# Autodesk Inventor assembly: 2.75 Omni AS, No Insert_CPY1
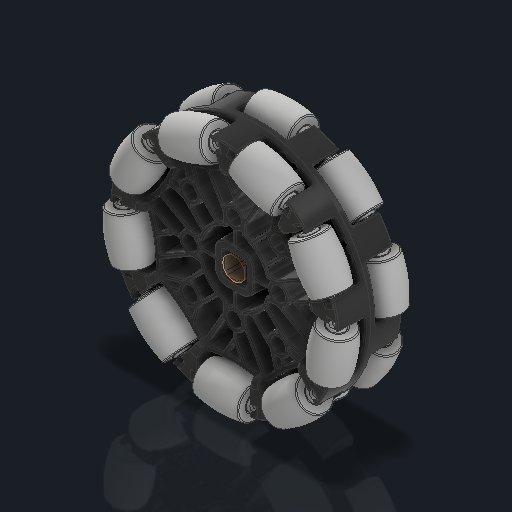
[picture p0: Inventor's stored thumbnail of the model, 512x512]
Saved by Autodesk Inventor 2023.2 (Build 272271030, 271C)
## iProperties
Created: 2022-08-02
Part Number: 2.75 Omni AS, No Insert_CPY1
Document SubType Name: Assembly
Designer: Michael
Author: ylu12
## Documents named in this file (2)
- C:\Users\black\OneDrive\Pictures\Documents\VEX CAD\VEX-CAD-Inventor-1.4.0\Motion\Wheels\Omni Wheel\2.75 Omni AS, No Insert_CPY1.iam
- C:\Users\black\OneDrive\Pictures\Documents\VEX CAD\VEX-CAD-Inventor-1.4.0\Motion\Wheels\Reference Files\2.75 Omni Antistatic_CPY1.ipt
## Components (1 placed, 1 different names)
1. 2.75 Omni Antistatic_CPY1:1 — Mate:8, Mate:7, Flush:4
## Relationships (3: Mate 2, Flush 1)
- Mate:8: 2.75 Omni Antistatic_CPY1:1
- Mate:7: 2.75 Omni Antistatic_CPY1:1
- Flush:4: 2.75 Omni Antistatic_CPY1:1
